# Autodesk Inventor assembly: LF
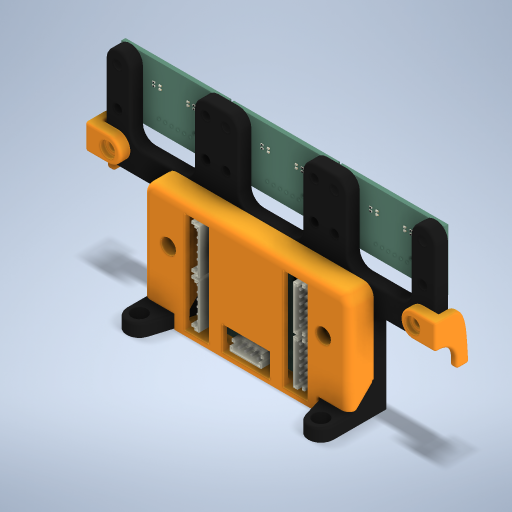
[picture p0: Inventor's stored thumbnail of the model, 512x512]
Saved by Autodesk Inventor 2023 (Build 270158000, 158)
## iProperties
Created: 2024-05-16
Part Number: LF
Document SubType Name: Assembly
Designer: kamil
Author: kamil
## Documents named in this file (7)
- C:\Users\kamil\Documents\PROJECTS - repos\ModBot---Projekt-Zespolowy\mechanics\LF.iam
- C:\Users\kamil\Documents\PROJECTS - repos\ModBot---Projekt-Zespolowy\mechanics\STEP\Hub LF.ipt
- C:\Users\kamil\Documents\PROJECTS - repos\ModBot---Projekt-Zespolowy\mechanics\STEP\Moduł LF.ipt
- C:\Users\kamil\Documents\PROJECTS - repos\ModBot---Projekt-Zespolowy\mechanics\lacznik.ipt
- C:\Users\kamil\Documents\PROJECTS - repos\ModBot---Projekt-Zespolowy\mechanics\pokrywa.ipt
- C:\Users\kamil\Documents\PROJECTS - repos\ModBot---Projekt-Zespolowy\mechanics\podpora.ipt
- C:\Users\kamil\Documents\PROJECTS - repos\ModBot---Projekt-Zespolowy\mechanics\podpora_MIR.ipt
## Components (8 placed, 6 different names)
1. Hub LF:1 — Zestawiające:3, Równoległe:6, Równoległe:7
2. Moduł LF:1 — Równoległe:1, Równoległe:2, Zestawiające:1, Równoległe:3, Zestawiające:2
3. Moduł LF:2 — Równoległe:1, Równoległe:2, Zestawiające:1, Równoległe:4, Równoległe:5
4. Moduł LF:3 — Równoległe:3, Równoległe:4, Zestawiające:2
5. lacznik:1 — Równoległe:5, Zestawiające:3, Równoległe:6, Równoległe:7, Równoległe:8, Zestawiające:4, Zestawiające:5, Kątowe:1, Symetria:1
6. pokrywa:1 — Równoległe:8, Symetria:1
7. podpora:1 — Zestawiające:4, Zestawiające:5, Kątowe:1
8. podpora_MIR:1
## Relationships (15: Flush 8, Mate 5, Angle 1, Symmetry 1)
- Równoległe:1 [Flush]: Moduł LF:1 ↔ Moduł LF:2
- Równoległe:2 [Flush]: Moduł LF:1 ↔ Moduł LF:2
- Zestawiające:1 [Mate] (1 mm): Moduł LF:1 ↔ Moduł LF:2
- Równoległe:3 [Flush]: Moduł LF:1 ↔ Moduł LF:3
- Równoległe:4 [Flush]: Moduł LF:2 ↔ Moduł LF:3
- Zestawiające:2 [Mate] (1 mm): Moduł LF:1 ↔ Moduł LF:3
- Równoległe:5 [Flush]: Moduł LF:2 ↔ lacznik:1
- Zestawiające:3 [Mate] (2 mm): Hub LF:1 ↔ lacznik:1
- Równoległe:6 [Flush] (-16.5 mm): Hub LF:1 ↔ lacznik:1
- Równoległe:7 [Flush] (3 mm): Hub LF:1 ↔ lacznik:1
- Równoległe:8 [Flush]: lacznik:1 ↔ pokrywa:1
- Zestawiające:4 [Mate]: lacznik:1 ↔ podpora:1
- Zestawiające:5 [Mate]: lacznik:1 ↔ podpora:1
- Kątowe:1 [Angle] (180 deg): lacznik:1 ↔ podpora:1
- Symetria:1 [Symmetry]: lacznik:1 ↔ pokrywa:1
